# Autodesk Inventor assembly: servo with bracket v9
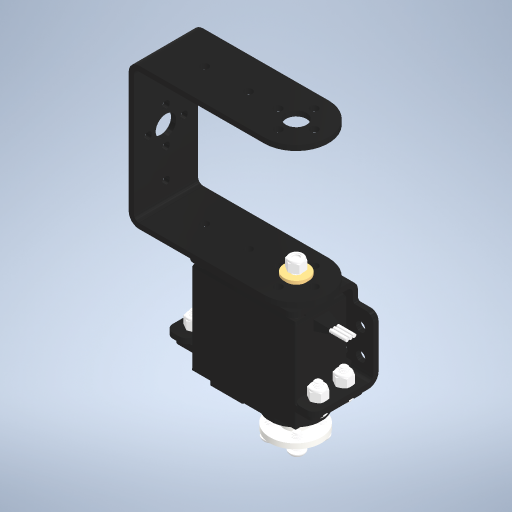
[picture p0: Inventor's stored thumbnail of the model, 512x512]
Saved by Autodesk Inventor 2024 (Build 280153000, 153)
## iProperties
Created: 2017-09-22
Part Number: servo with bracket v9
Document SubType Name: Assembly
Designer: ASUS
Sending System: Autodesk Translation Framework v6.1.1.50
Preprocessor: ST-DEVELOPER v16.13
Title: C:/Users/User/Desktop/servo with bracket v9.step
## Documents named in this file (8)
- C:\Users\ASUS\OneDrive\Dokumen\TUGAS\Servo with Bracket\servo with bracket 2.iam
- C:\Users\ASUS\OneDrive\Dokumen\TUGAS\Servo with Bracket\MG996 v1 v12.iam
- C:\Users\ASUS\OneDrive\Dokumen\TUGAS\Servo with Bracket\Servo Bracket - universal v10.iam
- C:\Users\ASUS\OneDrive\Dokumen\TUGAS\Servo with Bracket\M3x10.ipt
- C:\Users\ASUS\OneDrive\Dokumen\TUGAS\Servo with Bracket\M3 safe nut.ipt
- C:\Users\ASUS\OneDrive\Dokumen\TUGAS\Servo with Bracket\Servo Bracket - long U v3.iam
- C:\Users\ASUS\OneDrive\Dokumen\TUGAS\Servo with Bracket\brass brushing v1.iam
- C:\Users\ASUS\OneDrive\Dokumen\TUGAS\Servo with Bracket\screws and nuts.iam
## Components (7 placed, 7 different names)
1. MG996 v1 v12:1 [sub-assembly]
2. Servo Bracket - universal v10:1 [sub-assembly] — Mate:2
3. M3x10:1
4. M3 safe nut:1
5. Servo Bracket - long U v3:1 [sub-assembly] — Mate:1, Mate:2
6. brass brushing v1:1 [sub-assembly] — Mate:1
7. screws and nuts:1 [sub-assembly]
## Relationships (2: Mate 2)
- Mate:1: Servo Bracket - long U v3:1 ↔ brass brushing v1:1
- Mate:2: Servo Bracket - universal v10:1 ↔ Servo Bracket - long U v3:1
